# Autodesk Inventor assembly: mgse-memesat
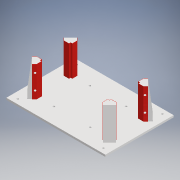
[picture p0: Inventor's stored thumbnail of the model, 180x180]
Saved by Autodesk Inventor 2022 (Build 260153000, 153)
## iProperties
Created: 2022-04-10
Part Number: mgse-memesat
Document SubType Name: Assembly
Designer: Cody
Author: Cody
## Documents named in this file (4)
- C:\$WorkingFolder\Engineering Data\MemeSat\MGSE\mgse-memesat.iam
- C:\$WorkingFolder\Engineering Data\MemeSat\MGSE\base.ipt
- C:\$WorkingFolder\Engineering Data\MemeSat\MGSE\tower.ipt
- C:\$WorkingFolder\Engineering Data\MemeSat\MGSE\guardv2.ipt
## Components (9 placed, 3 different names)
1. base:1 — Insert:1, Insert:2, Insert:3, Insert:4, Angle:1, Angle:2, Angle:3, Angle:4
2. tower:1 — Insert:1, Angle:1, Mate:1, Mate:2, Flush:1
3. tower:2 — Insert:2, Angle:2, Flush:2, Mate:3, Mate:4
4. tower:3 — Insert:3, Angle:3, Flush:3, Mate:5, Mate:9
5. tower:4 — Insert:4, Angle:4, Flush:4, Mate:6, Mate:7, Mate:8
6. guardv2:1 — Flush:3, Mate:5, Mate:9
7. guardv2:2 — Mate:1, Mate:2, Flush:1
8. guardv2:3 — Flush:4, Mate:6, Mate:7, Mate:8
9. guardv2:4 — Flush:2, Mate:3, Mate:4
## Relationships (21: Mate 9, Insert 4, Angle 4, Flush 4)
- Insert:1: base:1 ↔ tower:1
- Insert:2: base:1 ↔ tower:2
- Insert:3: base:1 ↔ tower:3
- Insert:4: base:1 ↔ tower:4
- Angle:1 (45 deg): base:1 ↔ tower:1
- Angle:2 (-45 deg): base:1 ↔ tower:2
- Angle:3 (45 deg): base:1 ↔ tower:3
- Angle:4 (-45 deg): base:1 ↔ tower:4
- Mate:1: tower:1 ↔ guardv2:2
- Mate:2: tower:1 ↔ guardv2:2
- Flush:1: tower:1 ↔ guardv2:2
- Flush:2: tower:2 ↔ guardv2:4
- Mate:3: tower:2 ↔ guardv2:4
- Mate:4: tower:2 ↔ guardv2:4
- Flush:3: tower:3 ↔ guardv2:1
- Mate:5: tower:3 ↔ guardv2:1
- Flush:4: tower:4 ↔ guardv2:3
- Mate:6: tower:4 ↔ guardv2:3
- Mate:7: tower:4 ↔ guardv2:3
- Mate:8: tower:4 ↔ guardv2:3
- Mate:9: tower:3 ↔ guardv2:1
